# Autodesk Inventor assembly: Сборка1
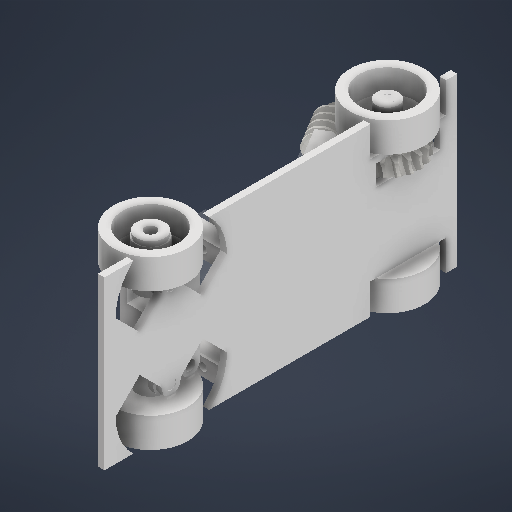
[picture p0: Inventor's stored thumbnail of the model, 512x512]
Saved by Autodesk Inventor 2026.2 (Build 302298000, 298)
## iProperties
Created: 2026-02-19
Part Number: Сборка1
Document SubType Name: Assembly
Designer: Leonid
Author: Leonid
## Documents named in this file (14)
- D:\Documents\Проекты\AutoBus\3Д модель\Рама\Сборка1.iam
- D:\Documents\Проекты\AutoBus\3Д модель\Рама\Малый сервопривод.ipt
- D:\Documents\Проекты\AutoBus\3Д модель\Рама\Рулевой толкатель на сервопривод.ipt
- D:\Documents\Проекты\AutoBus\3Д модель\Рама\Колесо переднее.ipt
- D:\Documents\Проекты\AutoBus\3Д модель\Рама\Рама1.ipt
- D:\Documents\Проекты\AutoBus\3Д модель\Рама\Кулак левый.ipt
- D:\Documents\Проекты\AutoBus\3Д модель\Рама\Штырь левый.ipt
- D:\Documents\Проекты\AutoBus\3Д модель\Рама\Тяга.ipt
- D:\Documents\Проекты\AutoBus\3Д модель\Рама\Кулак правый.ipt
- D:\Documents\Проекты\AutoBus\3Д модель\Рама\Штырь правый.ipt
- D:\Documents\Проекты\AutoBus\3Д модель\Рама\Мотор 17x8.ipt
- D:\Documents\Проекты\AutoBus\3Д модель\Рама\Сборка1\Мастер проектирования\Червячная передача8.iam
- D:\Documents\Проекты\AutoBus\3Д модель\Рама\Вал.ipt
- D:\Documents\Проекты\AutoBus\3Д модель\Рама\Колесо заднее.ipt
## Components (15 placed, 13 different names)
1. Рама1:1 — Цилиндрический:3, Совмещение:2, Заподлицо:2, Совмещение:12, Цилиндрический:16, Угол:1, Совмещение:13, Совмещение:15, Совмещение:16, Угол:2, Цилиндрический:19, Цилиндрический:21, Совмещение:19, Совмещение:20, Совмещение:21
2. Малый сервопривод:1 — Цилиндрический:11, Заподлицо:3, Совмещение:15, Совмещение:16
3. Кулак правый:1 — Цилиндрический:14, Совмещение:11, Совмещение:12, Цилиндрический:16, Цилиндрический:18, Заподлицо:7
4. Кулак левый:2 — Цилиндрический:3, Совмещение:2, Цилиндрический:4, Совмещение:4, Цилиндрический:13, Заподлицо:6
5. Тяга:1 — Цилиндрический:13, Касательность:1, Цилиндрический:14, Совмещение:13
6. Штырь правый:1 — Цилиндрический:17, Цилиндрический:18, Совмещение:14, Заподлицо:7
7. Штырь левый:2 — Цилиндрический:4, Цилиндрический:5, Совмещение:3, Заподлицо:6
8. Колесо переднее:1 — Совмещение:11, Цилиндрический:17, Совмещение:14
9. Колесо переднее:2 — Цилиндрический:5, Совмещение:3, Совмещение:4
10. Рулевой толкатель на сервопривод:1 — Цилиндрический:11, Заподлицо:3, Касательность:1, Заподлицо:2, Угол:1, Угол:2
11. Мотор 17x8:1 — Цилиндрический:20, Совмещение:17
12. Червячная передача:6 [sub-assembly] — Цилиндрический:19, Цилиндрический:20, Совмещение:17, Совмещение:21
13. Вал:1 — Цилиндрический:21, Цилиндрический:22, Заподлицо:8, Цилиндрический:23
14. Колесо заднее:1 — Цилиндрический:22, Совмещение:19, Заподлицо:8
15. Колесо заднее:2 — Цилиндрический:23, Совмещение:20
## Relationships (35: CylindricalJoint 14, Mate 13, Flush 5, Angle 2, Tangent 1)
- Цилиндрический:3 [CylindricalJoint]: Рама1:1 ↔ Кулак левый:2
- Совмещение:2 [Mate] (0.1 mm): Рама1:1 ↔ Кулак левый:2
- Заподлицо:2 [Flush] (-27.7 mm): Рама1:1 ↔ Рулевой толкатель на сервопривод:1
- Цилиндрический:4 [CylindricalJoint]: Кулак левый:2 ↔ Штырь левый:2
- Цилиндрический:5 [CylindricalJoint]: Штырь левый:2 ↔ Колесо переднее:2
- Совмещение:3 [Mate]: Штырь левый:2 ↔ Колесо переднее:2
- Совмещение:4 [Mate]: Кулак левый:2 ↔ Колесо переднее:2
- Цилиндрический:11 [CylindricalJoint]: Малый сервопривод:1 ↔ Рулевой толкатель на сервопривод:1
- Заподлицо:3 [Flush]: Малый сервопривод:1 ↔ Рулевой толкатель на сервопривод:1
- Цилиндрический:13 [CylindricalJoint]: Кулак левый:2 ↔ Тяга:1
- Касательность:1 [Tangent] (0.075 mm): Тяга:1 ↔ Рулевой толкатель на сервопривод:1
- Цилиндрический:14 [CylindricalJoint]: Кулак правый:1 ↔ Тяга:1
- Совмещение:11 [Mate]: Кулак правый:1 ↔ Колесо переднее:1
- Совмещение:12 [Mate] (0.1 mm): Рама1:1 ↔ Кулак правый:1
- Цилиндрический:16 [CylindricalJoint]: Рама1:1 ↔ Кулак правый:1
- Угол:1 [Angle] (38 deg): Рама1:1 ↔ Рулевой толкатель на сервопривод:1
- Совмещение:13 [Mate] (0.15 mm): Рама1:1 ↔ Тяга:1
- Заподлицо:6 [Flush]: Кулак левый:2 ↔ Штырь левый:2
- Цилиндрический:17 [CylindricalJoint]: Штырь правый:1 ↔ Колесо переднее:1
- Цилиндрический:18 [CylindricalJoint]: Кулак правый:1 ↔ Штырь правый:1
- Совмещение:14 [Mate]: Штырь правый:1 ↔ Колесо переднее:1
- Заподлицо:7 [Flush]: Кулак правый:1 ↔ Штырь правый:1
- Совмещение:15 [Mate]: Рама1:1 ↔ Малый сервопривод:1
- Совмещение:16 [Mate]: Рама1:1 ↔ Малый сервопривод:1
- Угол:2 [Angle] (0 deg): Рама1:1 ↔ Рулевой толкатель на сервопривод:1
- Цилиндрический:19 [CylindricalJoint]: Рама1:1 ↔ Червячная передача:6
- Цилиндрический:20 [CylindricalJoint]: Мотор 17x8:1 ↔ Червячная передача:6
- Совмещение:17 [Mate]: Мотор 17x8:1 ↔ Червячная передача:6
- Цилиндрический:21 [CylindricalJoint]: Рама1:1 ↔ Вал:1
- Цилиндрический:22 [CylindricalJoint]: Вал:1 ↔ Колесо заднее:1
- Совмещение:19 [Mate] (0.25 mm): Рама1:1 ↔ Колесо заднее:1
- Заподлицо:8 [Flush]: Вал:1 ↔ Колесо заднее:1
- Цилиндрический:23 [CylindricalJoint]: Вал:1 ↔ Колесо заднее:2
- Совмещение:20 [Mate] (0.25 mm): Рама1:1 ↔ Колесо заднее:2
- Совмещение:21 [Mate] (0.15 mm): Рама1:1 ↔ Червячная передача:6
